# Autodesk Inventor assembly: Montagem5
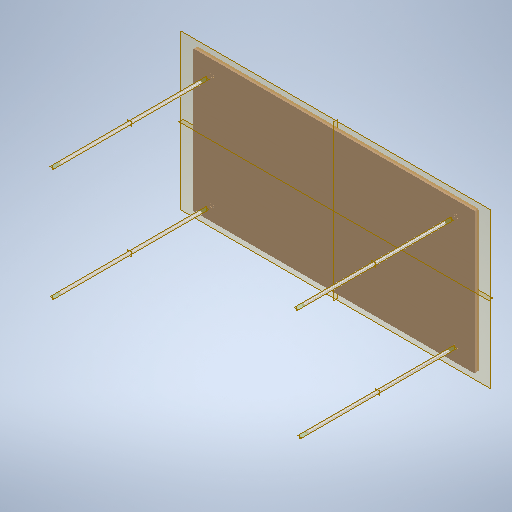
[picture p0: Inventor's stored thumbnail of the model, 512x512]
Saved by Autodesk Inventor 2025.2 (Build 292293000, 293)
## iProperties
Created: 2025-03-28
Part Number: Montagem5
Document SubType Name: Assembly
Designer: Formação
Author: Formação
## Documents named in this file (3)
- C:\Users\Formação\Documents\Inventor\NomeProjeto_2\Montagem5.iam
- C:\Users\Formação\Documents\Inventor\NomeProjeto_2\Peça9_mesa.ipt
- C:\Users\Formação\Documents\Inventor\NomeProjeto_2\Peça8_perna.ipt
## Components (5 placed, 2 different names)
1. Peça9_mesa:1 — Alinhado:1, Alinhado:2, Alinhado:3, Alinhado:4
2. Peça8_perna:1 — Alinhado:5, Coincidente:2, Simetria:1, Alinhado:6, Alinhado:7, Simetria:2, Alinhado:8, Alinhado:9
3. Peça8_perna:2 — Alinhado:7, Simetria:2, Alinhado:9, Simetria:4
4. Peça8_perna:4 — Simetria:1, Alinhado:6, Simetria:3
5. Peça8_perna:5 — Alinhado:8, Simetria:3, Simetria:4
## Relationships (14: Flush 9, Symmetry 4, Mate 1)
- Alinhado:1 [Flush]: Peça9_mesa:1
- Alinhado:2 [Flush]: Peça9_mesa:1
- Alinhado:3 [Flush]: Peça9_mesa:1
- Alinhado:4 [Flush]: Peça9_mesa:1
- Alinhado:5 [Flush] (-650 mm): Peça8_perna:1
- Coincidente:2 [Mate] (300 mm): Peça8_perna:1
- Simetria:1 [Symmetry]: Peça8_perna:1 ↔ Peça8_perna:4
- Alinhado:6 [Flush]: Peça8_perna:1 ↔ Peça8_perna:4
- Alinhado:7 [Flush]: Peça8_perna:1 ↔ Peça8_perna:2
- Simetria:2 [Symmetry]: Peça8_perna:1 ↔ Peça8_perna:2
- Alinhado:8 [Flush]: Peça8_perna:1 ↔ Peça8_perna:5
- Alinhado:9 [Flush]: Peça8_perna:1 ↔ Peça8_perna:2
- Simetria:3 [Symmetry]: Peça8_perna:4 ↔ Peça8_perna:5
- Simetria:4 [Symmetry]: Peça8_perna:2 ↔ Peça8_perna:5
